# Autodesk Inventor assembly: Joystick
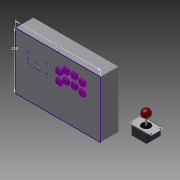
[picture p0: Inventor's stored thumbnail of the model, 180x180]
Saved by Autodesk Inventor 2013 (Build 170138000, 138)
## iProperties
Created: 2013-01-11
Part Number: Joystick
Document SubType Name: Assembly
Designer: mstine
Author: mstine
## Documents named in this file (5)
- C:\Users\mstine\Desktop\pewpew\assemblies\Joystick.iam
- C:\Users\mstine\Desktop\pewpew\parts\Body.ipt
- C:\Users\mstine\Desktop\pewpew\parts\Panel_top_2.ipt
- C:\Users\mstine\Desktop\pewpew\parts\OBSF-30-B_button.ipt
- C:\Users\mstine\Desktop\pewpew\parts\JLF-TP-8YT_joystick.ipt
## Components (11 placed, 4 different names)
1. Body:1 — Mate:1, Flush:1, Flush:2
2. TopPanel:1 — Mate:1, Flush:1, Flush:2, Tangent:1, Mate:2, Tangent:2, Mate:3, Tangent:3, Mate:4, Tangent:4, Mate:5, Tangent:5, Mate:6, Tangent:6, Mate:7, Tangent:7, Mate:8, Tangent:8, Mate:9
3. OBSF-30-B_button:1 — Tangent:1, Mate:2
4. OBSF-30-B_button:2 — Tangent:2, Mate:3
5. OBSF-30-B_button:3 — Tangent:4, Mate:5
6. OBSF-30-B_button:4 — Tangent:7, Mate:8
7. OBSF-30-B_button:5 — Tangent:6, Mate:7
8. OBSF-30-B_button:6 — Tangent:8, Mate:9
9. OBSF-30-B_button:7 — Tangent:5, Mate:6
10. OBSF-30-B_button:8 — Tangent:3, Mate:4
11. JLF-TP-8YT_joystick:1
## Relationships (19: Mate 9, Tangent 8, Flush 2)
- Mate:1: Body:1 ↔ TopPanel:1
- Flush:1: Body:1 ↔ TopPanel:1
- Flush:2: Body:1 ↔ TopPanel:1
- Tangent:1: TopPanel:1 ↔ OBSF-30-B_button:1
- Mate:2: TopPanel:1 ↔ OBSF-30-B_button:1
- Tangent:2: TopPanel:1 ↔ OBSF-30-B_button:2
- Mate:3: TopPanel:1 ↔ OBSF-30-B_button:2
- Tangent:3: TopPanel:1 ↔ OBSF-30-B_button:8
- Mate:4: TopPanel:1 ↔ OBSF-30-B_button:8
- Tangent:4: TopPanel:1 ↔ OBSF-30-B_button:3
- Mate:5: TopPanel:1 ↔ OBSF-30-B_button:3
- Tangent:5: TopPanel:1 ↔ OBSF-30-B_button:7
- Mate:6: TopPanel:1 ↔ OBSF-30-B_button:7
- Tangent:6: TopPanel:1 ↔ OBSF-30-B_button:5
- Mate:7: TopPanel:1 ↔ OBSF-30-B_button:5
- Tangent:7: TopPanel:1 ↔ OBSF-30-B_button:4
- Mate:8: TopPanel:1 ↔ OBSF-30-B_button:4
- Tangent:8: TopPanel:1 ↔ OBSF-30-B_button:6
- Mate:9: TopPanel:1 ↔ OBSF-30-B_button:6
